# Autodesk Inventor assembly: SS_5GL2_F_flat
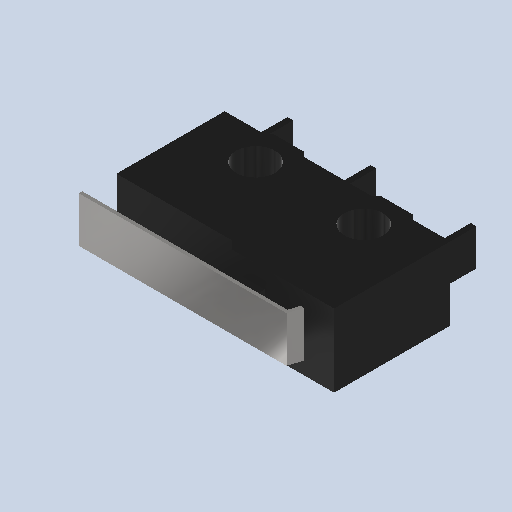
[picture p0: Inventor's stored thumbnail of the model, 512x512]
Saved by Autodesk Inventor 2022.3 (Build 263350000, 350)
## iProperties
Created: 2020-06-21
Part Number: SS_5GL2_F_flat
Document SubType Name: Assembly
Designer: Hagihara Yuya
Author: Hagihara Yuya
## Documents named in this file (3)
- C:\Users\YusukeKunita\Documents\GrabCAD\NHK2022\BasicParts\LimitSwitch\SS_5GL2_F_flat.iam
- C:\Users\YusukeKunita\Documents\GrabCAD\NHK2022\BasicParts\LimitSwitch\SS_5GL2_F_BASE.ipt
- C:\Users\YusukeKunita\Documents\GrabCAD\NHK2022\BasicParts\LimitSwitch\SS_5GL2_F_ACTUATOR_flat.ipt
## Components (2 placed, 2 different names)
1. SS_5GL2_F_BASE:1 — フラッシュ:1, メイト:1, 角度:1
2. SS_5GL2_F_ACTUATOR_flat:1 — フラッシュ:1, メイト:1, 角度:1
## Relationships (3: Flush 1, Mate 1, Angle 1)
- フラッシュ:1 [Flush] (1.2 mm): SS_5GL2_F_BASE:1 ↔ SS_5GL2_F_ACTUATOR_flat:1
- メイト:1 [Mate]: SS_5GL2_F_BASE:1 ↔ SS_5GL2_F_ACTUATOR_flat:1
- 角度:1 [Angle] (0 deg): SS_5GL2_F_BASE:1 ↔ SS_5GL2_F_ACTUATOR_flat:1
